# Autodesk Inventor assembly: Assembly2
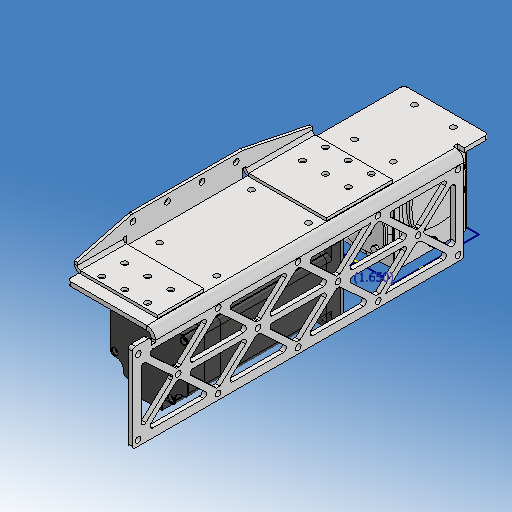
[picture p0: Inventor's stored thumbnail of the model, 512x512]
Saved by Autodesk Inventor 2025 (Build 290162000, 162)
## iProperties
Created: 2024-06-22
Part Number: Assembly2
Document SubType Name: Assembly
Designer: seene
Author: seene
## Documents named in this file (6)
- C:\Users\seene\Desktop\Stony Brook\SBRT\RCR_Dexter\Drive\TestRigs\Assembly2.iam
- C:\Users\seene\Desktop\Stony Brook\SBRT\RCR_Dexter\Drive\v1\StepperMotorStandOff.ipt
- C:\Users\seene\Desktop\Stony Brook\SBRT\RCR_Dexter\Drive\v1\34HS59-6004D-E1000 .ipt
- C:\Users\seene\Desktop\Stony Brook\SBRT\RCR_Dexter\Drive\QuintinCAD\NEMA34_gearbox_sheetMetaMount.ipt
- C:\Users\seene\Desktop\Stony Brook\SBRT\RCR_Dexter\Drive\v1\5887K172_Right-Angle Speed Reducer.ipt
- C:\Users\seene\Desktop\Stony Brook\SBRT\RCR_Dexter\Drive\v1\mainDriveSuppportBracket.ipt
## Components (5 placed, 5 different names)
1. StepperMotorStandOff:1 — Mate:1, Mate:2, Mate:3, Mate:4, Mate:5, Flush:1, Mate:6, Mate:7
2. 34HS59-6004D-E1000 :1 — Mate:1, Mate:2, Mate:3, Flush:1, Mate:6
3. NEMA34_gearbox_sheetMetaMount:1 — Mate:4, Mate:5, Mate:7, Mate:8, Mate:9, Mate:10, Mate:11, Mate:12, Mate:13
4. 5887K172_Right-Angle Speed Reducer:1 — Mate:8, Mate:9, Mate:10
5. mainDriveSuppportBracket:1 — Mate:11, Mate:12, Mate:13
## Relationships (14: Mate 13, Flush 1)
- Mate:1: StepperMotorStandOff:1 ↔ 34HS59-6004D-E1000 :1
- Mate:2: StepperMotorStandOff:1 ↔ 34HS59-6004D-E1000 :1
- Mate:3: StepperMotorStandOff:1 ↔ 34HS59-6004D-E1000 :1
- Mate:4: StepperMotorStandOff:1 ↔ NEMA34_gearbox_sheetMetaMount:1
- Mate:5: StepperMotorStandOff:1 ↔ NEMA34_gearbox_sheetMetaMount:1
- Flush:1: StepperMotorStandOff:1 ↔ 34HS59-6004D-E1000 :1
- Mate:6: StepperMotorStandOff:1 ↔ 34HS59-6004D-E1000 :1
- Mate:7: StepperMotorStandOff:1 ↔ NEMA34_gearbox_sheetMetaMount:1
- Mate:8: NEMA34_gearbox_sheetMetaMount:1 ↔ 5887K172_Right-Angle Speed Reducer:1
- Mate:9: NEMA34_gearbox_sheetMetaMount:1 ↔ 5887K172_Right-Angle Speed Reducer:1
- Mate:10: NEMA34_gearbox_sheetMetaMount:1 ↔ 5887K172_Right-Angle Speed Reducer:1
- Mate:11: NEMA34_gearbox_sheetMetaMount:1 ↔ mainDriveSuppportBracket:1
- Mate:12: NEMA34_gearbox_sheetMetaMount:1 ↔ mainDriveSuppportBracket:1
- Mate:13: NEMA34_gearbox_sheetMetaMount:1 ↔ mainDriveSuppportBracket:1
